# Autodesk Inventor assembly: pelican_electronics_asm
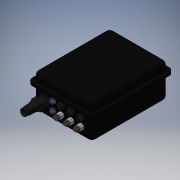
[picture p0: Inventor's stored thumbnail of the model, 180x180]
Saved by Autodesk Inventor 2017 SP1 (Build 210196100, 196)
## iProperties
Created: 2016-04-02
Part Number: pelican_electronics_asm
Document SubType Name: Assembly
Designer: hwasserb
Author: hwasserb
## Documents named in this file (18)
- C:\Users\Haden\Desktop\Charlie-CAD-Model\Robot Model\Pelican Case\Pelican Case.iam
- C:\Users\Haden\Desktop\Charlie-CAD-Model\Robot Model\Pelican Case\1400_BOTTOM.ipt
- C:\Users\Haden\Desktop\Charlie-CAD-Model\Robot Model\Pelican Case\BS2302.ipt
- C:\Users\Haden\Desktop\Charlie-CAD-Model\Robot Model\Pelican Case\15600-06-20.ipt
- C:\Users\Haden\Desktop\Charlie-CAD-Model\Robot Model\Pelican Case\TALON_SRX.ipt
- C:\Users\Haden\Desktop\Charlie-CAD-Model\Robot Model\Pelican Case\RJ45-PASSTHROUGH.ipt
- C:\Users\Haden\Desktop\Charlie-CAD-Model\Robot Model\Pelican Case\DT04-4P-L012.ipt
- C:\Users\Haden\Desktop\Charlie-CAD-Model\Robot Model\Pelican Case\DT06-4S.ipt
- C:\Users\Haden\Desktop\Charlie-CAD-Model\Robot Model\Pelican Case\WPUSBAX-MA1.ipt
- C:\Users\Haden\Desktop\Charlie-CAD-Model\Robot Model\Pelican Case\SK2-050B04.ipt
- C:\Users\Haden\Desktop\Charlie-CAD-Model\Robot Model\Pelican Case\SK6-050B04.ipt
- C:\Users\Haden\Desktop\Charlie-CAD-Model\Robot Model\Pelican Case\1400_TOP.ipt
- C:\Users\Haden\Desktop\Charlie-CAD-Model\Robot Model\Pelican Case\BOLT_10-32X1-1_4.ipt
- C:\Users\Haden\Desktop\Charlie-CAD-Model\Robot Model\Pelican Case\BOLT_10-32X1.ipt
- C:\Users\Haden\Desktop\Charlie-CAD-Model\Robot Model\Pelican Case\BOLT_8-32X1-3_8.ipt
- C:\Users\Haden\Desktop\Charlie-CAD-Model\Robot Model\Pelican Case\BOLT_8-32X3_4.ipt
- C:\Users\Haden\Desktop\Charlie-CAD-Model\Robot Model\Pelican Case\Interfacer\Interfacer.iam
- C:\Users\Haden\Desktop\Charlie-CAD-Model\Robot Model\Pelican Case\Netgear GS105 Enet Switch\Netgear GS105 Enet Switch.iam
## Components (49 placed, 17 different names)
1. 1400_BOTTOM:1 — Insert:1, Insert:2, Insert:3, Insert:4, Insert:5, Insert:6, Insert:7, Insert:8, Insert:9, Insert:10, Insert:11, Insert:12, Insert:13, Insert:14, Insert:15, Insert:16, Insert:17, Insert:18, Insert:19, Insert:20, Insert:21, Insert:22, Insert:23, Insert:24, Insert:25, Insert:26, Insert:27, Insert:28, Mate:1, Mate:2, Mate:3, Insert:49, Insert:50, Insert:51, Insert:52, Insert:53, Insert:54, Insert:55, Insert:56, Insert:57, Insert:58, Insert:59, Insert:60, Insert:61, Insert:62, Insert:63, Insert:64, Insert:65, Insert:66, Insert:67, Insert:68
2. BS2302:1 — Insert:15, Insert:16
3. 15600-06-20:1 — Insert:3, Insert:4
4. 15600-06-20:2 — Insert:5, Insert:6
5. TALON_SRX:1 — Insert:23, Insert:24
6. TALON_SRX:2 — Insert:19, Insert:20
7. RJ45-PASSTHROUGH:1
8. RJ45-PASSTHROUGH:2
9. RJ45-PASSTHROUGH:3
10. RJ45-PASSTHROUGH:4
11. DT04-4P-L012:1 — Insert:53, Insert:54
12. DT04-4P-L012:2 — Insert:51, Insert:52
13. DT04-4P-L012:3 — Insert:49, Insert:50
14. DT06-4S:1
15. DT06-4S:2
16. DT06-4S:3
17. WPUSBAX-MA1:1
18. WPUSBAX-MA1:2
19. SK2-050B04:1 — Insert:67, Insert:68
20. SK6-050B04:1
21. 1400_TOP:1
22. BOLT_10-32X1-1_4:1 — Insert:7
23. BOLT_10-32X1-1_4:2 — Insert:9
24. BOLT_10-32X1-1_4:3 — Insert:10
25. BOLT_10-32X1-1_4:4 — Insert:8
26. BOLT_10-32X1-1_4:5 — Insert:13
27. BOLT_10-32X1-1_4:6 — Insert:14
28. BOLT_10-32X1-1_4:7 — Insert:11
29. BOLT_10-32X1-1_4:8 — Insert:12
30. BOLT_10-32X1:1 — Insert:18
31. BOLT_10-32X1:2 — Insert:17
32. BOLT_8-32X1-3_8:1 — Insert:26
33. BOLT_8-32X1-3_8:2 — Insert:28
34. BOLT_8-32X1-3_8:3 — Insert:27
35. BOLT_8-32X1-3_8:4 — Insert:25
36. BOLT_8-32X3_4:1 — Insert:56
37. BOLT_8-32X3_4:2 — Insert:66
38. BOLT_8-32X3_4:3 — Insert:65
39. BOLT_8-32X3_4:4 — Insert:64
40. BOLT_8-32X3_4:5 — Insert:63
41. BOLT_8-32X3_4:6 — Insert:62
42. BOLT_8-32X3_4:7 — Insert:61
43. BOLT_8-32X3_4:8 — Insert:60
44. BOLT_8-32X3_4:9 — Insert:59
45. BOLT_8-32X3_4:10 — Insert:55
46. BOLT_8-32X3_4:11 — Insert:58
47. BOLT_8-32X3_4:12 — Insert:57
48. Interfacer:1 [sub-assembly] — Insert:1, Insert:2, Insert:21, Insert:22
49. Netgear GS105 Enet Switch:1 [sub-assembly] — Mate:1, Mate:2, Mate:3
## Relationships (51: Insert 48, Mate 3)
- Insert:1: 1400_BOTTOM:1 ↔ Interfacer:1
- Insert:2: 1400_BOTTOM:1 ↔ Interfacer:1
- Insert:3: 1400_BOTTOM:1 ↔ 15600-06-20:1
- Insert:4: 1400_BOTTOM:1 ↔ 15600-06-20:1
- Insert:5: 1400_BOTTOM:1 ↔ 15600-06-20:2
- Insert:6: 1400_BOTTOM:1 ↔ 15600-06-20:2
- Insert:7: 1400_BOTTOM:1 ↔ BOLT_10-32X1-1_4:1
- Insert:8: 1400_BOTTOM:1 ↔ BOLT_10-32X1-1_4:4
- Insert:9: 1400_BOTTOM:1 ↔ BOLT_10-32X1-1_4:2
- Insert:10: 1400_BOTTOM:1 ↔ BOLT_10-32X1-1_4:3
- Insert:11: 1400_BOTTOM:1 ↔ BOLT_10-32X1-1_4:7
- Insert:12: 1400_BOTTOM:1 ↔ BOLT_10-32X1-1_4:8
- Insert:13: 1400_BOTTOM:1 ↔ BOLT_10-32X1-1_4:5
- Insert:14: 1400_BOTTOM:1 ↔ BOLT_10-32X1-1_4:6
- Insert:15: 1400_BOTTOM:1 ↔ BS2302:1
- Insert:16: 1400_BOTTOM:1 ↔ BS2302:1
- Insert:17: 1400_BOTTOM:1 ↔ BOLT_10-32X1:2
- Insert:18: 1400_BOTTOM:1 ↔ BOLT_10-32X1:1
- Insert:19: 1400_BOTTOM:1 ↔ TALON_SRX:2
- Insert:20: 1400_BOTTOM:1 ↔ TALON_SRX:2
- Insert:21: 1400_BOTTOM:1 ↔ Interfacer:1
- Insert:22: 1400_BOTTOM:1 ↔ Interfacer:1
- Insert:23: 1400_BOTTOM:1 ↔ TALON_SRX:1
- Insert:24: 1400_BOTTOM:1 ↔ TALON_SRX:1
- Insert:25: 1400_BOTTOM:1 ↔ BOLT_8-32X1-3_8:4
- Insert:26: 1400_BOTTOM:1 ↔ BOLT_8-32X1-3_8:1
- Insert:27: 1400_BOTTOM:1 ↔ BOLT_8-32X1-3_8:3
- Insert:28: 1400_BOTTOM:1 ↔ BOLT_8-32X1-3_8:2
- Mate:1: 1400_BOTTOM:1 ↔ Netgear GS105 Enet Switch:1
- Mate:2: 1400_BOTTOM:1 ↔ Netgear GS105 Enet Switch:1
- Mate:3: 1400_BOTTOM:1 ↔ Netgear GS105 Enet Switch:1
- Insert:49: 1400_BOTTOM:1 ↔ DT04-4P-L012:3
- Insert:50: 1400_BOTTOM:1 ↔ DT04-4P-L012:3
- Insert:51: 1400_BOTTOM:1 ↔ DT04-4P-L012:2
- Insert:52: 1400_BOTTOM:1 ↔ DT04-4P-L012:2
- Insert:53: 1400_BOTTOM:1 ↔ DT04-4P-L012:1
- Insert:54: 1400_BOTTOM:1 ↔ DT04-4P-L012:1
- Insert:55: 1400_BOTTOM:1 ↔ BOLT_8-32X3_4:10
- Insert:56: 1400_BOTTOM:1 ↔ BOLT_8-32X3_4:1
- Insert:57: 1400_BOTTOM:1 ↔ BOLT_8-32X3_4:12
- Insert:58: 1400_BOTTOM:1 ↔ BOLT_8-32X3_4:11
- Insert:59: 1400_BOTTOM:1 ↔ BOLT_8-32X3_4:9
- Insert:60: 1400_BOTTOM:1 ↔ BOLT_8-32X3_4:8
- Insert:61: 1400_BOTTOM:1 ↔ BOLT_8-32X3_4:7
- Insert:62: 1400_BOTTOM:1 ↔ BOLT_8-32X3_4:6
- Insert:63: 1400_BOTTOM:1 ↔ BOLT_8-32X3_4:5
- Insert:64: 1400_BOTTOM:1 ↔ BOLT_8-32X3_4:4
- Insert:65: 1400_BOTTOM:1 ↔ BOLT_8-32X3_4:3
- Insert:66: 1400_BOTTOM:1 ↔ BOLT_8-32X3_4:2
- Insert:67: 1400_BOTTOM:1 ↔ SK2-050B04:1
- Insert:68: 1400_BOTTOM:1 ↔ SK2-050B04:1
